# Autodesk Inventor assembly: Oring-probe-flange-with-GV
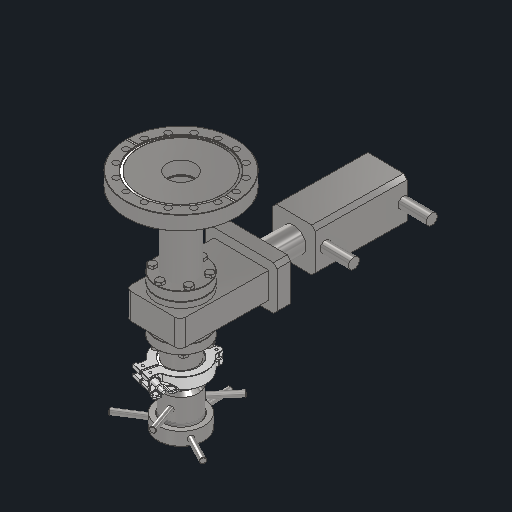
[picture p0: Inventor's stored thumbnail of the model, 512x512]
Saved by Autodesk Inventor 2027.1 (Build 311270010, 270A)
## iProperties
Created: 2024-05-30
Part Number: Oring-probe-flange-with-GV
Document SubType Name: Assembly
Designer: kuzmin
Author: kuzmin
## Documents named in this file (9)
- C:\Users\queezz\Dropbox\Drawings\PIHTI\Plasma Vessel\Oring-probe-flange-with-GV.iam
- C:\Users\queezz\Dropbox\Drawings\PIHTI\ContentCenter\CF-parts\CF-Flanges\CF_152-70.ipt
- C:\Users\queezz\Dropbox\Drawings\PIHTI\ContentCenter\CF-parts\CF70-nipple\CF70-nipple.iam
- C:\Users\queezz\Dropbox\Drawings\PIHTI\ContentCenter\CF-parts\CF70-gate-valve\Gatevalve_70_pneumatic.iam
- C:\Users\queezz\Dropbox\Drawings\PIHTI\ContentCenter\CF-KF-adapters\ICF70_to_KF40.ipt
- C:\Users\queezz\Dropbox\Drawings\PIHTI\PALP\OringFixture.iam
- C:\Users\queezz\Dropbox\Drawings\PIHTI\ContentCenter\NW\NW40_clamp.ipt
- C:\Users\queezz\Dropbox\Drawings\PIHTI\ContentCenter\NW\NW40_viton_centering_ring.ipt
- C:\Users\queezz\Dropbox\Drawings\PIHTI\ContentCenter\Fastners\M6x20-HexCS.ipt
## Components (25 placed, 8 different names)
1. CF_152-70:1 — Rotational:3, Mate:2
2. CF70-nipple:1 [sub-assembly] — Rotational:3, Mate:2, Rigid:4, Rigid:5, Rigid:6, Rigid:7, Rigid:8, Rigid:9, Rigid:10, Rigid:11, Rigid:12, Rigid:13, Rigid:14, Rotational:4
3. Gatevalve_70_pneumatic:1 [sub-assembly]
4. ICF70_to_KF40:1 — Rigid:15, Rigid:16, Rigid:17, Rigid:18, Rigid:19, Rotational:5
5. OringFixture:1 [sub-assembly]
6. NW40_clamp:1
7. NW40_viton_centering_ring:1
8. DIN EN 24017 M6 x 20:1 — Rigid:4
9. DIN EN 24017 M6 x 20:2 — Rigid:5
10. DIN EN 24017 M6 x 20:3 — Rigid:6
11. DIN EN 24017 M6 x 20:4 — Rigid:8
12. DIN EN 24017 M6 x 20:5 — Rigid:9
13. DIN EN 24017 M6 x 20:6 — Rigid:7
14. DIN EN 24017 M6 x 20:7 — Rotational:5
15. DIN EN 24017 M6 x 20:8 — Rigid:12
16. DIN EN 24017 M6 x 20:9 — Rigid:11
17. DIN EN 24017 M6 x 20:10 — Rigid:10
18. DIN EN 24017 M6 x 20:11 — Rigid:13
19. DIN EN 24017 M6 x 20:12 — Rigid:14
20. DIN EN 24017 M6 x 20:13 — Rigid:18
21. DIN EN 24017 M6 x 20:14 — Rigid:17
22. DIN EN 24017 M6 x 20:15 — Rigid:15
23. DIN EN 24017 M6 x 20:16 — Rigid:16
24. DIN EN 24017 M6 x 20:17 — Rotational:4
25. DIN EN 24017 M6 x 20:18 — Rigid:19
## Relationships (26: WeldJoint 18, RevoluteJoint 5, Mate 2, Flush 1)
- Rotational:3 [RevoluteJoint]: CF_152-70:1 ↔ CF70-nipple:1
- [RevoluteJoint]: CF70-nipple:1 ↔ Gatevalve_70_pneumatic:1
- [RevoluteJoint]: Gatevalve_70_pneumatic:1 ↔ ICF70_to_KF40:1
- [WeldJoint]: ICF70_to_KF40:1 ↔ NW40_viton_centering_ring:1
- [WeldJoint]: OringFixture:1 ↔ NW40_viton_centering_ring:1
- [Mate]: NW40_clamp:1 ↔ NW40_viton_centering_ring:1
- [Flush]: NW40_clamp:1 ↔ NW40_viton_centering_ring:1
- Mate:2: CF_152-70:1 ↔ CF70-nipple:1
- Rigid:4 [WeldJoint]: CF70-nipple:1 ↔ DIN EN 24017 M6 x 20:1
- Rigid:5 [WeldJoint]: CF70-nipple:1 ↔ DIN EN 24017 M6 x 20:2
- Rigid:6 [WeldJoint]: CF70-nipple:1 ↔ DIN EN 24017 M6 x 20:3
- Rigid:7 [WeldJoint]: CF70-nipple:1 ↔ DIN EN 24017 M6 x 20:6
- Rigid:8 [WeldJoint]: CF70-nipple:1 ↔ DIN EN 24017 M6 x 20:4
- Rigid:9 [WeldJoint]: CF70-nipple:1 ↔ DIN EN 24017 M6 x 20:5
- Rigid:10 [WeldJoint]: CF70-nipple:1 ↔ DIN EN 24017 M6 x 20:10
- Rigid:11 [WeldJoint]: CF70-nipple:1 ↔ DIN EN 24017 M6 x 20:9
- Rigid:12 [WeldJoint]: CF70-nipple:1 ↔ DIN EN 24017 M6 x 20:8
- Rigid:13 [WeldJoint]: CF70-nipple:1 ↔ DIN EN 24017 M6 x 20:11
- Rigid:14 [WeldJoint]: CF70-nipple:1 ↔ DIN EN 24017 M6 x 20:12
- Rigid:15 [WeldJoint]: ICF70_to_KF40:1 ↔ DIN EN 24017 M6 x 20:15
- Rigid:16 [WeldJoint]: ICF70_to_KF40:1 ↔ DIN EN 24017 M6 x 20:16
- Rigid:17 [WeldJoint]: ICF70_to_KF40:1 ↔ DIN EN 24017 M6 x 20:14
- Rigid:18 [WeldJoint]: ICF70_to_KF40:1 ↔ DIN EN 24017 M6 x 20:13
- Rigid:19 [WeldJoint]: ICF70_to_KF40:1 ↔ DIN EN 24017 M6 x 20:18
- Rotational:4 [RevoluteJoint]: CF70-nipple:1 ↔ DIN EN 24017 M6 x 20:17
- Rotational:5 [RevoluteJoint]: ICF70_to_KF40:1 ↔ DIN EN 24017 M6 x 20:7
